# Autodesk Inventor assembly: gears
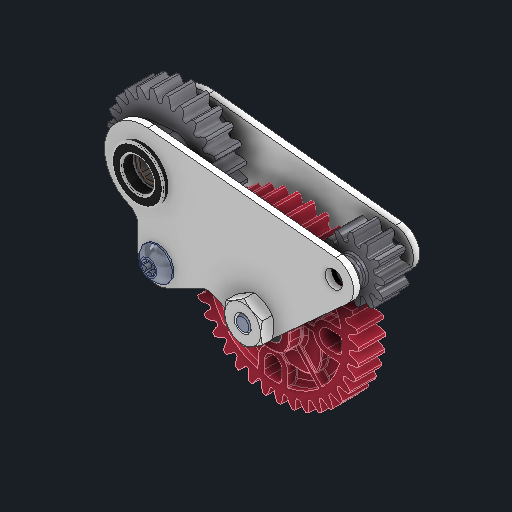
[picture p0: Inventor's stored thumbnail of the model, 512x512]
Saved by Autodesk Inventor 2024 (Build 280153000, 153)
## iProperties
Created: 2023-08-16
Part Number: gears
Document SubType Name: Assembly
Designer: avere
Author: avere
## Documents named in this file (13)
- D:\vex_robotics\hardware\cad\scrap_v0.1\catapult\gears.iam
- D:\vex_robotics\hardware\cad\scrap_v0.1\catapult\custom_parts\gear_gusset.ipt
- D:\vex_robotics\hardware\cad\VEX-CAD-Inventor-1.41\Motion\Shaft HS\HS Bushing 0.1250.ipt
- D:\vex_robotics\hardware\cad\scrap_v0.1\catapult\custom_parts\half_cut_24.ipt
- D:\vex_robotics\hardware\cad\VEX-CAD-Inventor-1.41\Motion\Gears\LS 12T Gear Steel.ipt
- D:\vex_robotics\hardware\cad\VEX-CAD-Inventor-1.41\Structure\Hardware\Screw Steel - Star\SScrew Star Smooth .750.ipt
- D:\vex_robotics\hardware\cad\VEX-CAD-Inventor-1.41\Structure\Hardware\Nut Nylon\Nut Nylon - White.ipt
- D:\vex_robotics\hardware\cad\scrap_v0.1\catapult\custom_parts\half_cut_36t.ipt
- D:\vex_robotics\hardware\cad\VEX-CAD-Inventor-1.41\Structure\Standoff\Standoff .50.ipt
- D:\vex_robotics\hardware\cad\VEX-CAD-Inventor-1.41\Structure\Hardware\Screw Steel - Star\SScrew Star Smooth .290.ipt
- D:\cad\VEX-CAD-Inventor-1.41\Structure\Hardware\Screw Steel - Star.ipt
- D:\cad\VEX-CAD-Inventor-1.41\Structure\Hardware\Nut Nylon.ipt
- D:\cad\VEX-CAD-Inventor-1.41\Structure\Standoff.ipt
## Components (12 placed, 9 different names)
1. gear_gusset:1 — Insert:1, Insert:5, Insert:6, Insert:7, Insert:10, Insert:12
2. HS Bushing 0.1250:1 — Insert:1, Insert:4
3. gear_gusset:2 — Insert:2, Insert:8, Insert:9, Insert:11
4. HS Bushing 0.1250:2 — Insert:2
5. half_cut_24:1 — Insert:4
6. LS 12T Gear Steel:1 — Insert:5
7. SScrew Star Smooth .750:1 — Insert:7
8. Nut Nylon - White:1 — Insert:8
9. half_cut_36t:1 — Insert:6
10. Standoff .50:1 — Insert:9, Insert:10
11. SScrew Star Smooth .290:2 — Insert:11
12. SScrew Star Smooth .290:3 — Insert:12
## Relationships (11: Insert 11)
- Insert:1: gear_gusset:1 ↔ HS Bushing 0.1250:1
- Insert:2: gear_gusset:2 ↔ HS Bushing 0.1250:2
- Insert:4: HS Bushing 0.1250:1 ↔ half_cut_24:1
- Insert:5 (1.5875 mm): gear_gusset:1 ↔ LS 12T Gear Steel:1
- Insert:6: gear_gusset:1 ↔ half_cut_36t:1
- Insert:7: gear_gusset:1 ↔ SScrew Star Smooth .750:1
- Insert:8: gear_gusset:2 ↔ Nut Nylon - White:1
- Insert:9: gear_gusset:2 ↔ Standoff .50:1
- Insert:10: gear_gusset:1 ↔ Standoff .50:1
- Insert:11: gear_gusset:2 ↔ SScrew Star Smooth .290:2
- Insert:12: gear_gusset:1 ↔ SScrew Star Smooth .290:3
